# Autodesk Inventor assembly: LeftGantryMount
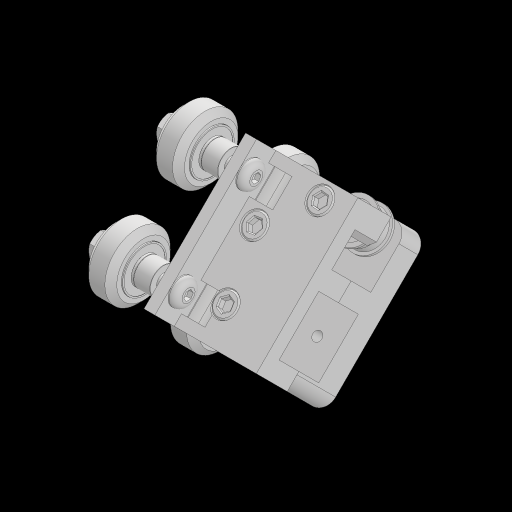
[picture p0: Inventor's stored thumbnail of the model, 512x512]
Saved by Autodesk Inventor 2023 (Build 270158000, 158)
## iProperties
Created: 2023-07-18
Part Number: LeftGantryMount
Document SubType Name: Assembly
Designer: tandu
Author: tandu
## Documents named in this file (7)
- C:\Users\tandu\Documents\GrabCAD\Custom Conveyor Belt 3D Printer\References\Roller based conveyor belt 3d printer\LeftGantryMount.iam
- C:\Users\tandu\Documents\GrabCAD\Custom Conveyor Belt 3D Printer\References\Roller based conveyor belt 3d printer\RollerVersionGates_2GT_20T_Toothed_Idler_Vychoz¡.ipt
- C:\Users\tandu\Documents\GrabCAD\Custom Conveyor Belt 3D Printer\References\Roller based conveyor belt 3d printer\RollerVersiongantry_mount_left_bottom_v2.ipt
- C:\Users\tandu\Documents\GrabCAD\Custom Conveyor Belt 3D Printer\References\Roller based conveyor belt 3d printer\RollerVersionF695 Bearing.step.ipt
- C:\Users\tandu\Documents\GrabCAD\Custom Conveyor Belt 3D Printer\References\Roller based conveyor belt 3d printer\RollerVersiongantry_mount_left_top_v2.ipt
- C:\Users\tandu\Documents\GrabCAD\Custom Conveyor Belt 3D Printer\References\Roller based conveyor belt 3d printer\RollerVersionM5x40.ipt
- C:\Users\tandu\Documents\GrabCAD\Custom Conveyor Belt 3D Printer\References\Roller based conveyor belt 3d printer\RollerVersionSVWB.iam
## Components (12 placed, 6 different names)
1. RollerVersionGates_2GT_20T_Toothed_Idler_Vychoz¡:1 — Insert:8
2. RollerVersiongantry_mount_left_bottom_v2:1 — Insert:3, Insert:4, Insert:11, Mate:1
3. RollerVersionF695 Bearing.step:1 — Insert:9, Insert:10
4. RollerVersionF695 Bearing.step:2 — Insert:10
5. RollerVersiongantry_mount_left_top_v2:1 — Insert:1, Insert:2, Insert:5, Insert:6, Insert:7, Insert:8, Insert:9, Insert:11, Mate:1
6. RollerVersionM5x40:1 — Insert:7
7. RollerVersionM5x40:2 — Insert:6
8. RollerVersionM5x40:3 — Insert:5
9. RollerVersionSVWB:1 [sub-assembly] — Insert:2
10. RollerVersionSVWB:2 [sub-assembly] — Insert:1
11. RollerVersionSVWB:3 [sub-assembly] — Insert:4
12. RollerVersionSVWB:4 [sub-assembly] — Insert:3
## Relationships (12: Insert 11, Mate 1)
- Insert:1: RollerVersiongantry_mount_left_top_v2:1 ↔ RollerVersionSVWB:2
- Insert:2: RollerVersiongantry_mount_left_top_v2:1 ↔ RollerVersionSVWB:1
- Insert:3: RollerVersiongantry_mount_left_bottom_v2:1 ↔ RollerVersionSVWB:4
- Insert:4: RollerVersiongantry_mount_left_bottom_v2:1 ↔ RollerVersionSVWB:3
- Insert:5: RollerVersiongantry_mount_left_top_v2:1 ↔ RollerVersionM5x40:3
- Insert:6: RollerVersiongantry_mount_left_top_v2:1 ↔ RollerVersionM5x40:2
- Insert:7: RollerVersiongantry_mount_left_top_v2:1 ↔ RollerVersionM5x40:1
- Insert:8: RollerVersionGates_2GT_20T_Toothed_Idler_Vychoz¡:1 ↔ RollerVersiongantry_mount_left_top_v2:1
- Insert:9: RollerVersionF695 Bearing.step:1 ↔ RollerVersiongantry_mount_left_top_v2:1
- Insert:10: RollerVersionF695 Bearing.step:1 ↔ RollerVersionF695 Bearing.step:2
- Insert:11: RollerVersiongantry_mount_left_bottom_v2:1 ↔ RollerVersiongantry_mount_left_top_v2:1
- Mate:1: RollerVersiongantry_mount_left_bottom_v2:1 ↔ RollerVersiongantry_mount_left_top_v2:1
